# Autodesk Inventor assembly: UFO
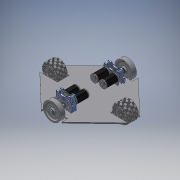
[picture p0: Inventor's stored thumbnail of the model, 180x180]
Saved by Autodesk Inventor 2018 (Build 220112000, 112)
## iProperties
Created: 2019-01-03
Part Number: UFO
Document SubType Name: Assembly
Designer: Gabriel
Author: Gabriel
## Documents named in this file (5)
- C:\Users\Gabriel\Documents\GitHub\2019CAD\Gab Drivebase Proto\UFO.iam
- C:\Users\Gabriel\Documents\GitHub\2019CAD\Gab Drivebase Proto\Wood Base.ipt
- C:\Users\Gabriel\Documents\GitHub\2019CAD\Summer Drivebase\6_Omni-Directional_Wheel_217-2585.ipt
- C:\Users\Gabriel\Documents\GitHub\2019CAD\Summer Drivebase\6in Colson Assem.iam
- C:\Users\Gabriel\Documents\GitHub\2019CAD\Summer Drivebase\Gearbox Assem.iam
## Components (9 placed, 4 different names)
1. Wood Base:1
2. 6_Omni-Directional_Wheel_217-2585:1
3. 6_Omni-Directional_Wheel_217-2585:2
4. 6_Omni-Directional_Wheel_217-2585:3
5. 6_Omni-Directional_Wheel_217-2585:4
6. 6in Colson Assem:1 [sub-assembly] — Mate:1, Mate:2
7. 6in Colson Assem:2 [sub-assembly] — Mate:3, Mate:4
8. Gearbox Assem:1 [sub-assembly] — Mate:1, Mate:2
9. Gearbox Assem:2 [sub-assembly] — Mate:3, Mate:4
## Relationships (4: Mate 4)
- Mate:1: 6in Colson Assem:1 ↔ Gearbox Assem:1
- Mate:2: 6in Colson Assem:1 ↔ Gearbox Assem:1
- Mate:3: 6in Colson Assem:2 ↔ Gearbox Assem:2
- Mate:4: 6in Colson Assem:2 ↔ Gearbox Assem:2
